# Autodesk Inventor assembly: MECANISMO DE COMPACTADO
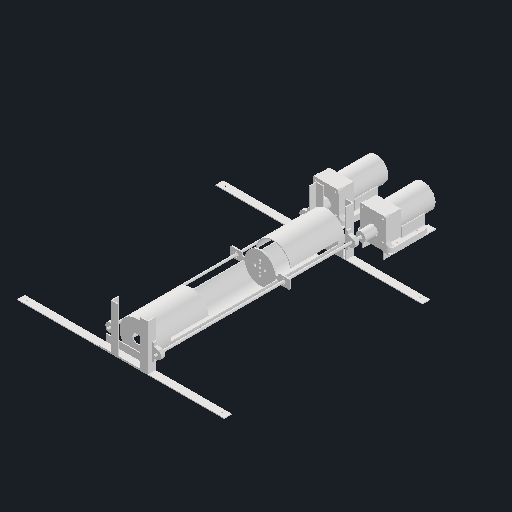
[picture p0: Inventor's stored thumbnail of the model, 512x512]
Saved by Autodesk Inventor 2024.3 (Build 283343000, 343)
## iProperties
Created: 2024-05-26
Part Number: MECANISMO DE COMPACTADO
Document SubType Name: Assembly
Designer: Jhuliams
Author: Jhuliams
## Documents named in this file (22)
- C:\Users\Niler\OneDrive\Escritorio\RECICLADOR\RECICLADOR_MODELO_3D\MECANISMO DE COMPACTADO\MECANISMO DE COMPACTADO.iam
- C:\Users\Niler\OneDrive\Escritorio\RECICLADOR\RECICLADOR_MODELO_3D\MECANISMO DE COMPACTADO\GUIA_DE_OBJETO.ipt
- C:\Users\Niler\OneDrive\Escritorio\RECICLADOR\RECICLADOR_MODELO_3D\MECANISMO DE COMPACTADO\TAPA QUE DESPLAZA CON TORNILLOS.ipt
- C:\Users\Niler\OneDrive\Escritorio\RECICLADOR\RECICLADOR_MODELO_3D\MECANISMO DE COMPACTADO\TUERCA DE HUSILLO.ipt
- C:\Users\Niler\OneDrive\Escritorio\RECICLADOR\RECICLADOR_MODELO_3D\MECANISMO DE COMPACTADO\TORNILLO DEPOTENCIA.ipt
- C:\Users\Niler\OneDrive\Escritorio\RECICLADOR\RECICLADOR_MODELO_3D\MECANISMO DE COMPACTADO\ACOPLE HELICOIDAL.ipt
- C:\Users\Niler\OneDrive\Escritorio\RECICLADOR\RECICLADOR_MODELO_3D\MECANISMO DE COMPACTADO\MOTOR DC.ipt
- C:\Users\Niler\OneDrive\Escritorio\RECICLADOR\RECICLADOR_MODELO_3D\MECANISMO DE COMPACTADO\RODAMIENTO DE TORNILLO.ipt
- C:\Users\Niler\OneDrive\Escritorio\RECICLADOR\RECICLADOR_MODELO_3D\MECANISMO DE COMPACTADO\PLETINA PARA GUIA CILINDRICA.ipt
- C:\Users\Niler\OneDrive\Escritorio\RECICLADOR\RECICLADOR_MODELO_3D\MECANISMO DE COMPACTADO\SOPORTE DEL MOTOR.ipt
- C:\Users\Niler\OneDrive\Escritorio\RECICLADOR\RECICLADOR_MODELO_3D\MECANISMO DE COMPACTADO\SOPORTE LATERAL DE GUIA CILINDRICA.ipt
- C:\Users\Niler\OneDrive\Escritorio\RECICLADOR\RECICLADOR_MODELO_3D\MECANISMO DE COMPACTADO\SOPORTE LATERAL DE GUIA CILINDRICA_MIR.ipt
- C:\Users\Niler\OneDrive\Escritorio\RECICLADOR\RECICLADOR_MODELO_3D\MECANISMO DE COMPACTADO\RODAMIENTO DE TORNILLO_MIR.ipt
- C:\Users\Niler\OneDrive\Escritorio\RECICLADOR\RECICLADOR_MODELO_3D\MECANISMO DE COMPACTADO\SOPORTE LATERAL DE GUIA CILINDRICA_MIR1.ipt
- C:\Users\Niler\OneDrive\Escritorio\RECICLADOR\RECICLADOR_MODELO_3D\MECANISMO DE COMPACTADO\RODAMIENTO DE TORNILLO_MIR1.ipt
- C:\Users\Niler\OneDrive\Escritorio\RECICLADOR\RECICLADOR_MODELO_3D\MECANISMO DE COMPACTADO\SOPORTE LATERAL DE GUIA CILINDRICA_MIR2.ipt
- C:\Users\Niler\OneDrive\Escritorio\RECICLADOR\RECICLADOR_MODELO_3D\MECANISMO DE COMPACTADO\RODAMIENTO DE TORNILLO_MIR_MIR.ipt
- C:\Users\Niler\OneDrive\Escritorio\RECICLADOR\RECICLADOR_MODELO_3D\MECANISMO DE COMPACTADO\SOPORTE LATERAL DE GUIA CILINDRICA_MIR1_MIR.ipt
- C:\Users\Niler\OneDrive\Escritorio\RECICLADOR\RECICLADOR_MODELO_3D\MECANISMO DE COMPACTADO\ACOPLE HELICOIDAL_MIR.ipt
- C:\Users\Niler\OneDrive\Escritorio\RECICLADOR\RECICLADOR_MODELO_3D\MECANISMO DE COMPACTADO\MOTOR DC_MIR.ipt
- C:\Users\Niler\OneDrive\Escritorio\RECICLADOR\RECICLADOR_MODELO_3D\MECANISMO DE COMPACTADO\SOPORTE DEL MOTOR_MIR.ipt
- C:\Users\Niler\OneDrive\Escritorio\RECICLADOR\RECICLADOR_MODELO_3D\MECANISMO DE COMPACTADO\SOPORTE LATERAL DE GUIA CILINDRICA_MIR3.ipt
## Components (28 placed, 21 different names)
1. PLETINA PARA GUIA CILINDRICA:1 — Mate:22, Flush:3, Mate:24, Flush:4, Flush:7, Flush:13, Flush:15, Mate:37
2. GUIA_DE_OBJETO:1 — Mate:6, Mate:7, Mate:8, Flush:2, Mate:21, Tangent:1, Mate:29, Tangent:2
3. TORNILLO DEPOTENCIA:1 — Mate:9, Mate:16, Flush:1, Mate:23, Mate:27, Flush:12, Mate:38, Mate:39
4. TORNILLO DEPOTENCIA:2 — Mate:10, Mate:15, Flush:1, Mate:34, Mate:35
5. TAPA QUE DESPLAZA CON TORNILLOS:1 — Mate:6, Mate:7, Mate:8, Mate:9, Mate:10, Mate:17, Mate:18, Mate:19, Mate:20
6. TUERCA DE HUSILLO:1 — Mate:16, Mate:17, Mate:20
7. TUERCA DE HUSILLO:2 — Mate:15, Mate:18, Mate:19
8. SOPORTE LATERAL DE GUIA CILINDRICA:1 — Flush:2, Mate:21, Tangent:1, Mate:22, Flush:3
9. SOPORTE LATERAL DE GUIA CILINDRICA_MIR:1 — Mate:29, Tangent:2, Mate:31, Flush:8
10. RODAMIENTO DE TORNILLO:1 — Mate:23, Mate:25, Flush:6, Flush:12
11. SOPORTE LATERAL DE GUIA CILINDRICA:2 — Mate:24, Mate:25, Flush:4, Flush:6
12. RODAMIENTO DE TORNILLO_MIR:1 — Mate:26, Flush:5, Mate:27
13. SOPORTE LATERAL DE GUIA CILINDRICA_MIR1:1 — Mate:26, Flush:5, Mate:30, Flush:9, Flush:22
14. PLETINA PARA GUIA CILINDRICA:2 — Flush:7, Mate:30, Mate:31, Flush:8, Flush:9, Flush:13, Mate:36, Flush:14, Mate:43, Flush:22
15. RODAMIENTO DE TORNILLO_MIR1:1 — Flush:10, Mate:32, Mate:35
16. SOPORTE LATERAL DE GUIA CILINDRICA_MIR2:1 — Flush:10, Mate:32, Flush:15, Mate:37
17. RODAMIENTO DE TORNILLO_MIR_MIR:1 — Flush:11, Mate:33, Mate:34
18. SOPORTE LATERAL DE GUIA CILINDRICA_MIR1_MIR:1 — Flush:11, Mate:33, Mate:36, Flush:14
19. ACOPLE HELICOIDAL:1 — Mate:38, Mate:39, Mate:40, Mate:41
20. MOTOR DC:1 — Mate:40, Mate:41, Mate:42, Flush:16, Flush:17
21. SOPORTE DEL MOTOR:1 — Mate:42, Flush:16, Flush:17, Mate:43, Mate:44, Flush:18, Flush:19, Mate:45, Flush:20, Flush:21
22. SOPORTE LATERAL DE GUIA CILINDRICA:3 — Mate:44, Flush:18, Flush:19
23. SOPORTE LATERAL DE GUIA CILINDRICA:4 — Mate:45, Flush:20, Flush:21
24. ACOPLE HELICOIDAL_MIR:1 — Mate:46, Mate:47
25. MOTOR DC_MIR:1 — Mate:46, Mate:47, Flush:23, Flush:24, Mate:48
26. SOPORTE DEL MOTOR_MIR:1 — Flush:23, Flush:24, Mate:48, Flush:25, Flush:26, Mate:49, Flush:27, Flush:28, Mate:50
27. SOPORTE LATERAL DE GUIA CILINDRICA_MIR3:1 — Flush:25, Flush:26, Mate:49
28. SOPORTE LATERAL DE GUIA CILINDRICA_MIR3:2 — Flush:27, Flush:28, Mate:50
## Relationships (70: Mate 40, Flush 28, Tangent 2)
- Mate:6: GUIA_DE_OBJETO:1 ↔ TAPA QUE DESPLAZA CON TORNILLOS:1
- Mate:7 (1 mm): GUIA_DE_OBJETO:1 ↔ TAPA QUE DESPLAZA CON TORNILLOS:1
- Mate:8 (1 mm): GUIA_DE_OBJETO:1 ↔ TAPA QUE DESPLAZA CON TORNILLOS:1
- Mate:9: TORNILLO DEPOTENCIA:1 ↔ TAPA QUE DESPLAZA CON TORNILLOS:1
- Mate:10: TORNILLO DEPOTENCIA:2 ↔ TAPA QUE DESPLAZA CON TORNILLOS:1
- Mate:15: TORNILLO DEPOTENCIA:2 ↔ TUERCA DE HUSILLO:2
- Mate:16: TORNILLO DEPOTENCIA:1 ↔ TUERCA DE HUSILLO:1
- Mate:17: TAPA QUE DESPLAZA CON TORNILLOS:1 ↔ TUERCA DE HUSILLO:1
- Mate:18: TAPA QUE DESPLAZA CON TORNILLOS:1 ↔ TUERCA DE HUSILLO:2
- Mate:19: TAPA QUE DESPLAZA CON TORNILLOS:1 ↔ TUERCA DE HUSILLO:2
- Mate:20: TAPA QUE DESPLAZA CON TORNILLOS:1 ↔ TUERCA DE HUSILLO:1
- Flush:1: TORNILLO DEPOTENCIA:1 ↔ TORNILLO DEPOTENCIA:2
- Flush:2 (48.325 mm): GUIA_DE_OBJETO:1 ↔ SOPORTE LATERAL DE GUIA CILINDRICA:1
- Mate:21: GUIA_DE_OBJETO:1 ↔ SOPORTE LATERAL DE GUIA CILINDRICA:1
- Tangent:1 (-7.5 mm): GUIA_DE_OBJETO:1 ↔ SOPORTE LATERAL DE GUIA CILINDRICA:1
- Mate:22: PLETINA PARA GUIA CILINDRICA:1 ↔ SOPORTE LATERAL DE GUIA CILINDRICA:1
- Flush:3: PLETINA PARA GUIA CILINDRICA:1 ↔ SOPORTE LATERAL DE GUIA CILINDRICA:1
- Mate:23: TORNILLO DEPOTENCIA:1 ↔ RODAMIENTO DE TORNILLO:1
- Mate:24: PLETINA PARA GUIA CILINDRICA:1 ↔ SOPORTE LATERAL DE GUIA CILINDRICA:2
- Mate:25: RODAMIENTO DE TORNILLO:1 ↔ SOPORTE LATERAL DE GUIA CILINDRICA:2
- Flush:4: PLETINA PARA GUIA CILINDRICA:1 ↔ SOPORTE LATERAL DE GUIA CILINDRICA:2
- Mate:26: RODAMIENTO DE TORNILLO_MIR:1 ↔ SOPORTE LATERAL DE GUIA CILINDRICA_MIR1:1
- Flush:5: RODAMIENTO DE TORNILLO_MIR:1 ↔ SOPORTE LATERAL DE GUIA CILINDRICA_MIR1:1
- Mate:27: TORNILLO DEPOTENCIA:1 ↔ RODAMIENTO DE TORNILLO_MIR:1
- Flush:6: RODAMIENTO DE TORNILLO:1 ↔ SOPORTE LATERAL DE GUIA CILINDRICA:2
- Mate:29: GUIA_DE_OBJETO:1 ↔ SOPORTE LATERAL DE GUIA CILINDRICA_MIR:1
- Tangent:2 (-107.5 mm): GUIA_DE_OBJETO:1 ↔ SOPORTE LATERAL DE GUIA CILINDRICA_MIR:1
- Flush:7: PLETINA PARA GUIA CILINDRICA:1 ↔ PLETINA PARA GUIA CILINDRICA:2
- Mate:30: SOPORTE LATERAL DE GUIA CILINDRICA_MIR1:1 ↔ PLETINA PARA GUIA CILINDRICA:2
- Mate:31: SOPORTE LATERAL DE GUIA CILINDRICA_MIR:1 ↔ PLETINA PARA GUIA CILINDRICA:2
- Flush:8: SOPORTE LATERAL DE GUIA CILINDRICA_MIR:1 ↔ PLETINA PARA GUIA CILINDRICA:2
- Flush:9: SOPORTE LATERAL DE GUIA CILINDRICA_MIR1:1 ↔ PLETINA PARA GUIA CILINDRICA:2
- Flush:10: RODAMIENTO DE TORNILLO_MIR1:1 ↔ SOPORTE LATERAL DE GUIA CILINDRICA_MIR2:1
- Mate:32: RODAMIENTO DE TORNILLO_MIR1:1 ↔ SOPORTE LATERAL DE GUIA CILINDRICA_MIR2:1
- Flush:11: RODAMIENTO DE TORNILLO_MIR_MIR:1 ↔ SOPORTE LATERAL DE GUIA CILINDRICA_MIR1_MIR:1
- Mate:33: RODAMIENTO DE TORNILLO_MIR_MIR:1 ↔ SOPORTE LATERAL DE GUIA CILINDRICA_MIR1_MIR:1
- Flush:12 (10 mm): TORNILLO DEPOTENCIA:1 ↔ RODAMIENTO DE TORNILLO:1
- Flush:13: PLETINA PARA GUIA CILINDRICA:1 ↔ PLETINA PARA GUIA CILINDRICA:2
- Mate:34: TORNILLO DEPOTENCIA:2 ↔ RODAMIENTO DE TORNILLO_MIR_MIR:1
- Mate:35: TORNILLO DEPOTENCIA:2 ↔ RODAMIENTO DE TORNILLO_MIR1:1
- Mate:36: PLETINA PARA GUIA CILINDRICA:2 ↔ SOPORTE LATERAL DE GUIA CILINDRICA_MIR1_MIR:1
- Flush:14: PLETINA PARA GUIA CILINDRICA:2 ↔ SOPORTE LATERAL DE GUIA CILINDRICA_MIR1_MIR:1
- Flush:15: PLETINA PARA GUIA CILINDRICA:1 ↔ SOPORTE LATERAL DE GUIA CILINDRICA_MIR2:1
- Mate:37: PLETINA PARA GUIA CILINDRICA:1 ↔ SOPORTE LATERAL DE GUIA CILINDRICA_MIR2:1
- Mate:38 (-20 mm): TORNILLO DEPOTENCIA:1 ↔ ACOPLE HELICOIDAL:1
- Mate:39: TORNILLO DEPOTENCIA:1 ↔ ACOPLE HELICOIDAL:1
- Mate:40: ACOPLE HELICOIDAL:1 ↔ MOTOR DC:1
- Mate:41 (10 mm): ACOPLE HELICOIDAL:1 ↔ MOTOR DC:1
- Mate:42: MOTOR DC:1 ↔ SOPORTE DEL MOTOR:1
- Flush:16 (-2.5 mm): MOTOR DC:1 ↔ SOPORTE DEL MOTOR:1
- Flush:17 (-2.5 mm): MOTOR DC:1 ↔ SOPORTE DEL MOTOR:1
- Mate:43 (15 mm): PLETINA PARA GUIA CILINDRICA:2 ↔ SOPORTE DEL MOTOR:1
- Mate:44: SOPORTE DEL MOTOR:1 ↔ SOPORTE LATERAL DE GUIA CILINDRICA:3
- Flush:18: SOPORTE DEL MOTOR:1 ↔ SOPORTE LATERAL DE GUIA CILINDRICA:3
- Flush:19: SOPORTE DEL MOTOR:1 ↔ SOPORTE LATERAL DE GUIA CILINDRICA:3
- Mate:45: SOPORTE DEL MOTOR:1 ↔ SOPORTE LATERAL DE GUIA CILINDRICA:4
- Flush:20: SOPORTE DEL MOTOR:1 ↔ SOPORTE LATERAL DE GUIA CILINDRICA:4
- Flush:21: SOPORTE DEL MOTOR:1 ↔ SOPORTE LATERAL DE GUIA CILINDRICA:4
- Flush:22 (250 mm): SOPORTE LATERAL DE GUIA CILINDRICA_MIR1:1 ↔ PLETINA PARA GUIA CILINDRICA:2
- Mate:46 (10 mm): ACOPLE HELICOIDAL_MIR:1 ↔ MOTOR DC_MIR:1
- Mate:47: ACOPLE HELICOIDAL_MIR:1 ↔ MOTOR DC_MIR:1
- Flush:23 (-2.5 mm): MOTOR DC_MIR:1 ↔ SOPORTE DEL MOTOR_MIR:1
- Flush:24 (-2.5 mm): MOTOR DC_MIR:1 ↔ SOPORTE DEL MOTOR_MIR:1
- Mate:48: MOTOR DC_MIR:1 ↔ SOPORTE DEL MOTOR_MIR:1
- Flush:25: SOPORTE DEL MOTOR_MIR:1 ↔ SOPORTE LATERAL DE GUIA CILINDRICA_MIR3:1
- Flush:26: SOPORTE DEL MOTOR_MIR:1 ↔ SOPORTE LATERAL DE GUIA CILINDRICA_MIR3:1
- Mate:49: SOPORTE DEL MOTOR_MIR:1 ↔ SOPORTE LATERAL DE GUIA CILINDRICA_MIR3:1
- Flush:27: SOPORTE DEL MOTOR_MIR:1 ↔ SOPORTE LATERAL DE GUIA CILINDRICA_MIR3:2
- Flush:28: SOPORTE DEL MOTOR_MIR:1 ↔ SOPORTE LATERAL DE GUIA CILINDRICA_MIR3:2
- Mate:50: SOPORTE DEL MOTOR_MIR:1 ↔ SOPORTE LATERAL DE GUIA CILINDRICA_MIR3:2
